# Autodesk Inventor assembly: B30037_MIR
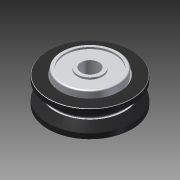
[picture p0: Inventor's stored thumbnail of the model, 180x180]
Saved by Autodesk Inventor 2014 (Build 180170000, 170)
## iProperties
Created: 2012-01-16
Part Number: B30037_MIR
Description: Dual Bearing V Wheel Kit (assembly)
Vendor: custom
Document SubType Name: Assembly
Designer: Edward
Stock Number: B30037_ASM
Mass: 3.05191 g
Surface Area: 39.551 cm^2
Volume: 2.4421 cm^3
Density: 1.24971 g/cm^3
Author: ERF
## Documents named in this file (4)
- C:\Users\Edward\Desktop\Shapeoko_v2.0\B30037_MIR.iam
- C:\Users\Edward\Desktop\Shapeoko_v2.0\B17021_MIR.ipt
- C:\Users\Edward\Desktop\Shapeoko_v2.0\BEARING_5_16_5_MIR.ipt
- C:\Users\Edward\Desktop\Shapeoko_v2.0\B18026_MIR.ipt
## Components (4 placed, 3 different names)
1. B17021_MIR:1 — Insert:3, Insert:1
2. BEARING_5_16_5_MIR:1 — Insert:3
3. BEARING_5_16_5_MIR:2 — Insert:1, Insert:4
4. B18026_MIR:1 — Insert:4
## Relationships (3: Insert 3)
- Insert:3: B17021_MIR:1 ↔ BEARING_5_16_5_MIR:1
- Insert:1: B17021_MIR:1 ↔ BEARING_5_16_5_MIR:2
- Insert:4: BEARING_5_16_5_MIR:2 ↔ B18026_MIR:1
